# Autodesk Inventor assembly: Print_Assembly_N_KATO_Z01-0281
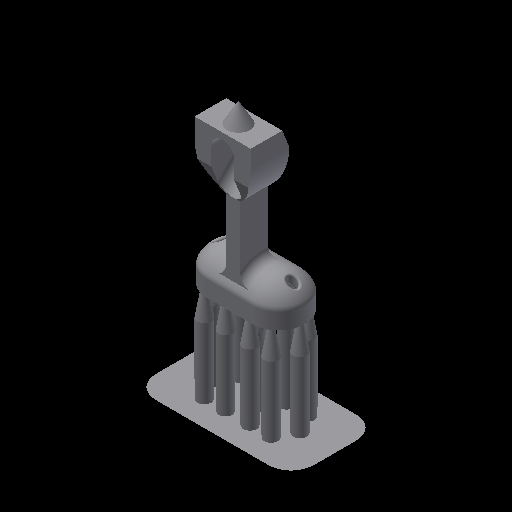
[picture p0: Inventor's stored thumbnail of the model, 512x512]
Saved by Autodesk Inventor 2026.2 (Build 302298010, 298A)
## iProperties
Manager: MANUTENÇÃO GUIFÕES - CP
Company: CP
Created: 2025-09-03
Part Number: Print_Assembly_N_KATO_Z01-0281
Project: 0.00 0000/00
Checked By: PMFIGUEIREDO
Engr Approved By: JSSILVA
Description: NOME DA PEÇA/MONTAGEM
Document SubType Name: Assembly
Designer: TPMIRANDA
Engineer: ISO 2768 - m K
Authority: Nº DESENHO PELO QUAL FOI SUBSITUIDO
Stock Number: 00000-000
Title: UME 3400
Subject: CAIXA, INTERIOR, SUPORTE,
Author: TPMIRANDA
Keywords: Caixa de comentários. Substituir texto, ou eliminar.
Comments: UQE2300 UQE2400 UTE2240 UDD9630 CARRUAGENS SIMAFE CARRUAGENS CAF CARRUAGENS ARCO
Revision Number: Nº DESENHO QUE SUBSTITUI
## Documents named in this file (5)
- C:\Users\tpmiranda\OneDrive - Comboios de Portugal EPE\Engate CNMF\Montagem\Print_Assembly_N_KATO_Z01-0281.iam
- C:\Users\tpmiranda\OneDrive - Comboios de Portugal EPE\Engate CNMF\Montagem\Stand.ipt
- C:\Users\tpmiranda\OneDrive - Comboios de Portugal EPE\Engate CNMF\Montagem\Base N.ipt
- C:\Users\tpmiranda\OneDrive - Comboios de Portugal EPE\Engate CNMF\Engates\Engate CNMF N KATO Z01-0281.ipt
- C:\Users\tpmiranda\OneDrive - Comboios de Portugal EPE\Engate CNMF\Engates\Engate CNMF N KATO Z01-0281\Engate CNMF PROFI-8.00.ipt
## Components (13 placed, 3 different names)
1. Base N:1 — Alinhado:13, Alinhado:14, Coincidente:24, Coincidente:2, Coincidente:20
2. Engate CNMF PROFI-8.00:1 — Coincidente:1, Alinhado:16, Coincidente:3, Alinhado:17, Coincidente:4, Coincidente:19, Alinhado:18, Coincidente:24
3. Stand:1 — Coincidente:1, Coincidente:2, Alinhado:17, Coincidente:4
4. Stand:2 — Coincidente:19, Coincidente:20, Alinhado:18
5. Stand:3
6. Stand:4
7. Stand:9
8. Stand:10
9. Stand:6
10. Stand:7
11. Stand:8
12. Stand:11
13. Stand:12
## Component patterns: (2 elements), (5 elements, first: Stand:2), Component Pattern 8:2 (5 elements)
## Relationships (12: Mate 7, Flush 5)
- Alinhado:13 [Flush]: Base N:1
- Alinhado:14 [Flush]: Base N:1
- Coincidente:24 [Mate]: Base N:1 ↔ Engate CNMF PROFI-8.00:1
- Coincidente:1 [Mate]: Engate CNMF PROFI-8.00:1 ↔ Stand:1
- Coincidente:2 [Mate]: Base N:1 ↔ Stand:1
- Alinhado:16 [Flush]: Engate CNMF PROFI-8.00:1
- Coincidente:3 [Mate] (-2.5 mm): Engate CNMF PROFI-8.00:1
- Alinhado:17 [Flush]: Engate CNMF PROFI-8.00:1 ↔ Stand:1
- Coincidente:4 [Mate]: Engate CNMF PROFI-8.00:1 ↔ Stand:1
- Coincidente:19 [Mate]: Engate CNMF PROFI-8.00:1 ↔ Stand:2
- Coincidente:20 [Mate]: Base N:1 ↔ Stand:2
- Alinhado:18 [Flush] (2.5 mm): Engate CNMF PROFI-8.00:1 ↔ Stand:2
